# Autodesk Inventor assembly: Sheathing_For_Back
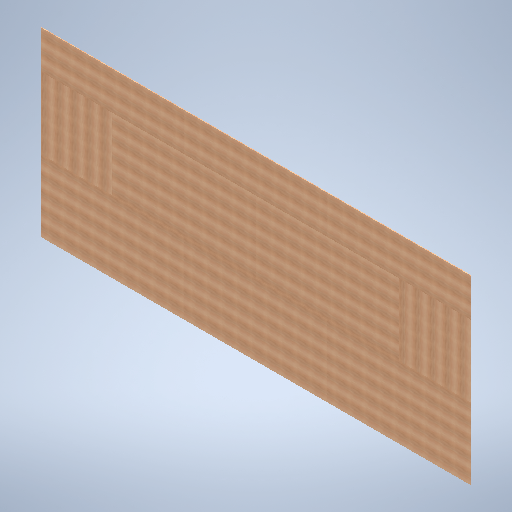
[picture p0: Inventor's stored thumbnail of the model, 512x512]
Saved by Autodesk Inventor 2025 (Build 290162010, 162A)
## iProperties
Created: 2024-10-03
Part Number: Sheathing_For_Back
Document SubType Name: Assembly
Designer: Tom
Author: Tom
## Documents named in this file (4)
- C:\Users\Tom\Documents\Inventor\Mobility\Additional_Building\Sheathing_For_Back.iam
- C:\Users\Tom\Documents\Inventor\Mobility\Additional_Building\OSB_For_Walls_With_Dimensions_48_x_96_Inches.ipt
- C:\Users\Tom\Documents\Inventor\Mobility\Additional_Building\OSB_For_Walls_With_Dimensions_48_x_48_Inches.ipt
- C:\Users\Tom\Documents\Inventor\Mobility\Additional_Building\OSB_For_Walls_With_Dimensions_25.5_x_96_Inches.ipt
## Components (10 placed, 3 different names)
1. OSB_For_Walls_With_Dimensions_48_x_96_Inches:1 — Mate:1, Mate:2, Flush:1, Mate:3, Flush:2, Flush:3, Flush:4
2. OSB_For_Walls_With_Dimensions_48_x_96_Inches:2 — Mate:4
3. OSB_For_Walls_With_Dimensions_48_x_96_Inches:3
4. OSB_For_Walls_With_Dimensions_48_x_96_Inches:4 — Mate:4, Mate:5, Flush:4, Mate:6
5. OSB_For_Walls_With_Dimensions_48_x_96_Inches:5
6. OSB_For_Walls_With_Dimensions_48_x_48_Inches:1 — Mate:3, Flush:2, Flush:3, Mate:5, Flush:5, Flush:6
7. OSB_For_Walls_With_Dimensions_48_x_48_Inches:2
8. OSB_For_Walls_With_Dimensions_25.5_x_96_Inches:1 — Mate:6, Flush:5, Flush:6
9. OSB_For_Walls_With_Dimensions_25.5_x_96_Inches:2
10. OSB_For_Walls_With_Dimensions_25.5_x_96_Inches:3
## Component patterns: (3 elements, first: OSB_For_Walls_With_Dimensions_48_x_96_Inches:1), (2 elements, first: OSB_For_Walls_With_Dimensions_48_x_96_Inches:4), (2 elements, first: OSB_For_Walls_With_Dimensions_48_x_48_Inches:1), (3 elements, first: OSB_For_Walls_With_Dimensions_25.5_x_96_Inches:1)
## Relationships (12: Mate 6, Flush 6)
- Mate:1: OSB_For_Walls_With_Dimensions_48_x_96_Inches:1
- Mate:2: OSB_For_Walls_With_Dimensions_48_x_96_Inches:1
- Flush:1: OSB_For_Walls_With_Dimensions_48_x_96_Inches:1
- Mate:3: OSB_For_Walls_With_Dimensions_48_x_96_Inches:1 ↔ OSB_For_Walls_With_Dimensions_48_x_48_Inches:1
- Flush:2: OSB_For_Walls_With_Dimensions_48_x_96_Inches:1 ↔ OSB_For_Walls_With_Dimensions_48_x_48_Inches:1
- Flush:3: OSB_For_Walls_With_Dimensions_48_x_96_Inches:1 ↔ OSB_For_Walls_With_Dimensions_48_x_48_Inches:1
- Mate:4: OSB_For_Walls_With_Dimensions_48_x_96_Inches:2 ↔ OSB_For_Walls_With_Dimensions_48_x_96_Inches:4
- Mate:5: OSB_For_Walls_With_Dimensions_48_x_96_Inches:4 ↔ OSB_For_Walls_With_Dimensions_48_x_48_Inches:1
- Flush:4: OSB_For_Walls_With_Dimensions_48_x_96_Inches:1 ↔ OSB_For_Walls_With_Dimensions_48_x_96_Inches:4
- Mate:6: OSB_For_Walls_With_Dimensions_48_x_96_Inches:4 ↔ OSB_For_Walls_With_Dimensions_25.5_x_96_Inches:1
- Flush:5: OSB_For_Walls_With_Dimensions_48_x_48_Inches:1 ↔ OSB_For_Walls_With_Dimensions_25.5_x_96_Inches:1
- Flush:6: OSB_For_Walls_With_Dimensions_48_x_48_Inches:1 ↔ OSB_For_Walls_With_Dimensions_25.5_x_96_Inches:1
